# Autodesk Inventor assembly: 左後脚ユニット5_MIR
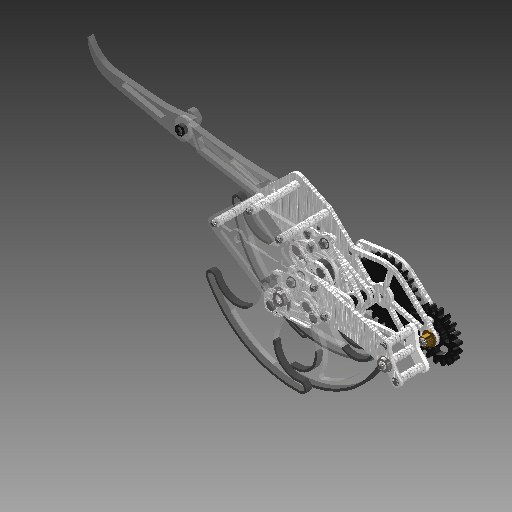
[picture p0: Inventor's stored thumbnail of the model, 512x512]
Saved by Autodesk Inventor 2020 (Build 240168000, 168)
## iProperties
Created: 2019-09-03
Part Number: 左後脚ユニット5_MIR
Document SubType Name: Assembly
Designer: 雪村
Mass: 251.015 g
Surface Area: 1556.42 cm^2
Volume: 120.818 cm^3
Density: 2.07763 g/cm^3
Author: 雪村
## Documents named in this file (29)
- C:\Users\white\Documents\SRDC\SRDC\Inventor_2017\2018年機体\2020年4年機体\右後脚ユニット5.iam
- C:\Users\white\Documents\SRDC\SRDC\Inventor_2017\2018年機体\2020年4年機体\脚内フレーム5_MIR2_MIR.ipt
- C:\Users\white\Documents\SRDC\SRDC\Inventor_2017\2018年機体\2020年4年機体\脚外フレーム5_MIR_MIR.ipt
- C:\Users\white\Documents\SRDC\SRDC\Inventor_2017\2018年機体\2020年4年機体\後脚ユニット締結パーツ5_MIR.ipt
- C:\Users\white\Documents\SRDC\SRDC\Inventor_2017\2018年機体\2020年4年機体\後脚ギアトレイン5.2_MIR.ipt
- C:\Users\white\Documents\SRDC\SRDC\Inventor_2017\2018年機体\2020年4年機体\後脚軸抑え1_MIR.ipt
- C:\Users\white\Documents\SRDC\SRDC\Inventor_2017\2018年機体\2020年4年機体\脚クランク1.iam
- C:\Users\white\Documents\SRDC\SRDC\Inventor_2017\2018年機体\2020年4年機体\ヘッケン＋揺動節2_MIR.iam
- C:\Users\white\Documents\SRDC\SRDC\Inventor_2017\2018年機体\2020年4年機体\歯車m2.z24.ipt
- C:\Users\white\Documents\SRDC\SRDC\Inventor_2017\2018年機体\2020年4年機体\脚最終段カム4.ipt
- C:\Users\white\Documents\SRDC\SRDC\Inventor_2017\2018年機体\パーツ\スペーサーm3,40.ipt
- C:\Users\white\Documents\SRDC\SRDC\Inventor_2017\2018年機体\パーツ\スペーサーm3,7.ipt
- C:\Users\white\Documents\SRDC\SRDC\Inventor_2017\2018年機体\2020年4年機体\歯車m2.z19.ipt
- C:\Users\white\Documents\SRDC\SRDC\Inventor_2017\2018年機体\パーツ\ベアリングフランジ付き0610.3t.ipt
- C:\Users\white\Documents\SRDC\SRDC\Inventor_2017\2018年機体\2020年4年機体\歯車m2.z25.ipt
- C:\Users\white\Documents\SRDC\SRDC\Inventor_2017\2018年機体\パーツ\オイレスフランジ付き06080512,1t ドライメット.ipt
- C:\Users\white\Documents\SRDC\SRDC\Inventor_2017\2018年機体\パーツ\スペーサーm3,6.ipt
- C:\Users\white\Documents\SRDC\SRDC\Inventor_2017\2018年機体\パーツ\ネジ鍋m3,12.ipt
- C:\Users\white\Documents\SRDC\SRDC\Inventor_2017\2018年機体\パーツ\オイレスフランジ付き12142003.ipt
- C:\Users\white\Documents\SRDC\SRDC\Inventor_2017\2018年機体\パーツ\スペーサーm3,4.ipt
- C:\Users\white\Documents\SRDC\SRDC\Inventor_2017\2018年機体\2020年4年機体\脚最終段カム3.ipt
- C:\Users\white\Documents\SRDC\SRDC\Inventor_2017\2018年機体\パーツ\ネジ皿m3,08.ipt
- C:\Users\white\Documents\SRDC\SRDC\Inventor_2017\2018年機体\パーツ\ネジ鍋m3,08.ipt
- C:\Users\white\Documents\SRDC\SRDC\Inventor_2017\2018年機体\パーツ\ネジ鍋m3,06.ipt
- C:\Users\white\Documents\SRDC\SRDC\Inventor_2017\2018年機体\パーツ\ネジ鍋m3,16.ipt
- C:\Users\white\Documents\SRDC\SRDC\Inventor_2017\2018年機体\2020年4年機体\後ウイング1_MIR.iam
- C:\Users\white\Documents\SRDC\SRDC\Inventor_2017\2018年機体\パーツ\スペーサーm3,20.ipt
- C:\Users\white\Documents\SRDC\SRDC\Inventor_2017\2018年機体\2020年4年機体\段ばね抑え2.ipt
- C:\Users\white\Documents\SRDC\SRDC\Inventor_2017\2018年機体\パーツ\スペーサーm3,5.ipt
## Components (75 placed, 28 different names)
1. 脚内フレーム5_MIR2_MIR:1 — メイト:1, メイト:2, メイト:3, メイト:4, 挿入:15, 挿入:16, 挿入:17, 挿入:18, 挿入:32, 挿入:33, 挿入:34, 挿入:36, 挿入:37, 挿入:38, 挿入:40, 挿入:41, 挿入:42, 挿入:44, 挿入:47, 挿入:48, 挿入:64, 挿入:70, 挿入:71, 挿入:72, 挿入:77
2. 脚外フレーム5_MIR_MIR:1 — 挿入:19, 挿入:20, 挿入:65, 挿入:66, 挿入:67, 挿入:68, 挿入:69, 挿入:90
3. 後脚ユニット締結パーツ5_MIR:1 — メイト:5, 挿入:73, 挿入:81, 挿入:82, 挿入:87, 挿入:88
4. 後脚ギアトレイン5.2_MIR:1 — 挿入:45, 挿入:46, 挿入:53, 挿入:54, 挿入:55, 挿入:62, 挿入:75
5. 後脚軸抑え1_MIR:1 — 挿入:49, 挿入:50, 挿入:56, 挿入:57, 挿入:63
6. 脚クランク1:1 [sub-assembly] — 挿入:29, メイト:6, 挿入:31, 挿入:89
7. ヘッケン＋揺動節2_MIR:1 [sub-assembly] — メイト:4
8. ヘッケン＋揺動節2_MIR:2 [sub-assembly] — メイト:3
9. ヘッケン＋揺動節2_MIR:3 [sub-assembly] — メイト:1
10. ヘッケン＋揺動節2_MIR:4 [sub-assembly] — メイト:2
11. 歯車m2.z24:1 — 挿入:30
12. 脚最終段カム4:1 — 挿入:58, 挿入:59, 挿入:60, 挿入:61
13. オイレスフランジ付き12142003:2 — メイト:7
14. スペーサーm3,40:1 — 挿入:18, 挿入:20, メイト:5
15. スペーサーm3,40:2 — 挿入:17
16. スペーサーm3,40:3 — 挿入:16
17. スペーサーm3,40:4 — 挿入:15, 挿入:19
18. スペーサーm3,7:2 — 挿入:34
19. スペーサーm3,7:3 — 挿入:38
20. スペーサーm3,7:4 — 挿入:44, 挿入:45
21. スペーサーm3,7:5 — 挿入:33, 挿入:46
22. 歯車m2.z19:1
23. ベアリングフランジ付き0610.3t:1
24. ベアリングフランジ付き0610.3t:2 — 挿入:41
25. 歯車m2.z25:1
26. ベアリングフランジ付き0610.3t:3 — 挿入:40
27. ベアリングフランジ付き0610.3t:4
28. オイレスフランジ付き06080512,1t ドライメット:1 — 挿入:75
29. オイレスフランジ付き06080512,1t ドライメット:2
30. スペーサーm3,6:1
31. スペーサーm3,6:2 — 挿入:42
32. ネジ鍋m3,12:1
33. ネジ鍋m3,12:2
34. スペーサーm3,6:3 — 挿入:37
35. スペーサーm3,6:4 — 挿入:36, 挿入:50
36. オイレスフランジ付き12142003:1 — 挿入:31, 挿入:32
37. 脚最終段カム3:1 — 挿入:29, メイト:6, 挿入:30, メイト:7
38. スペーサーm3,7:6 — 挿入:47
39. スペーサーm3,6:5 — 挿入:48, 挿入:49
40. ネジ鍋m3,12:3 — 挿入:53
41. ネジ鍋m3,12:4 — 挿入:55
42. ネジ鍋m3,12:5 — 挿入:62
43. ネジ鍋m3,12:6 — 挿入:54
44. ネジ鍋m3,12:7 — 挿入:63
45. ネジ鍋m3,12:8 — 挿入:56
46. ネジ鍋m3,12:9 — 挿入:57
47. ネジ皿m3,08:1 — 挿入:64
48. ネジ鍋m3,08:1 — 挿入:67
49. ネジ鍋m3,08:2 — 挿入:68
50. ネジ鍋m3,08:3 — 挿入:66
51. ネジ鍋m3,08:4 — 挿入:71
52. ネジ鍋m3,08:5 — 挿入:72
53. ネジ鍋m3,08:6 — 挿入:70, 挿入:76
54. ネジ鍋m3,08:7 — 挿入:69
55. ネジ鍋m3,06:1 — 挿入:65
56. ネジ鍋m3,16:1 — 挿入:61
57. ネジ鍋m3,16:2 — 挿入:59
58. ネジ鍋m3,16:3 — 挿入:60
59. ネジ鍋m3,16:4 — 挿入:58
60. スペーサーm3,4:1 — 挿入:73, 挿入:74, 挿入:86
61. ベアリングフランジ付き0610.3t:5 — 挿入:74
62. 後ウイング1_MIR:1 [sub-assembly] — 挿入:76, 正接:1
63. スペーサーm3,6:6 — 挿入:77, 正接:1
64. スペーサーm3,20:1 — 挿入:78, 挿入:82
65. スペーサーm3,20:2 — 挿入:79
66. スペーサーm3,20:3 — 挿入:80, 挿入:81
67. 段ばね抑え2:1 — 挿入:78, 挿入:79, 挿入:80, 挿入:83, 挿入:84, 挿入:85
68. ネジ鍋m3,08:8 — 挿入:84
69. ネジ鍋m3,08:9 — 挿入:83
70. ネジ鍋m3,08:10 — 挿入:85
71. ネジ鍋m3,12:10 — 挿入:86
72. ネジ皿m3,08:2 — 挿入:87
73. ネジ皿m3,08:3 — 挿入:88
74. ベアリングフランジ付き0610.3t:6 — 挿入:90
75. スペーサーm3,5:1 — 挿入:89
## Relationships (86: Insert 78, Mate 7, Tangent 1)
- [Insert] (0.5 mm): 脚クランク1:1 ↔ ヘッケン＋揺動節2_MIR:1
- [Insert] (0.5 mm): 脚クランク1:1 ↔ ヘッケン＋揺動節2_MIR:2
- [Insert] (0.5 mm): 脚クランク1:1 ↔ ヘッケン＋揺動節2_MIR:3
- [Insert] (0.5 mm): 脚クランク1:1 ↔ ヘッケン＋揺動節2_MIR:4
- [Insert]: 歯車m2.z24:1 ↔ 脚最終段カム4:1
- [Insert]: 歯車m2.z24:1 ↔ 脚最終段カム4:1
- [Insert]: 脚最終段カム4:1 ↔ オイレスフランジ付き12142003:2
- メイト:1 [Mate]: 脚内フレーム5_MIR2_MIR:1 ↔ ヘッケン＋揺動節2_MIR:3
- メイト:2 [Mate]: 脚内フレーム5_MIR2_MIR:1 ↔ ヘッケン＋揺動節2_MIR:4
- メイト:3 [Mate]: 脚内フレーム5_MIR2_MIR:1 ↔ ヘッケン＋揺動節2_MIR:2
- メイト:4 [Mate]: 脚内フレーム5_MIR2_MIR:1 ↔ ヘッケン＋揺動節2_MIR:1
- 挿入:15 [Insert]: 脚内フレーム5_MIR2_MIR:1 ↔ スペーサーm3,40:4
- 挿入:16 [Insert]: 脚内フレーム5_MIR2_MIR:1 ↔ スペーサーm3,40:3
- 挿入:17 [Insert]: 脚内フレーム5_MIR2_MIR:1 ↔ スペーサーm3,40:2
- 挿入:18 [Insert]: 脚内フレーム5_MIR2_MIR:1 ↔ スペーサーm3,40:1
- 挿入:19 [Insert]: 脚外フレーム5_MIR_MIR:1 ↔ スペーサーm3,40:4
- 挿入:20 [Insert]: 脚外フレーム5_MIR_MIR:1 ↔ スペーサーm3,40:1
- メイト:5 [Mate]: 後脚ユニット締結パーツ5_MIR:1 ↔ スペーサーm3,40:1
- [Insert]: 歯車m2.z19:1 ↔ ベアリングフランジ付き0610.3t:1
- [Insert]: 歯車m2.z19:1 ↔ ベアリングフランジ付き0610.3t:2
- [Insert]: 歯車m2.z25:1 ↔ ベアリングフランジ付き0610.3t:3
- [Insert]: 歯車m2.z25:1 ↔ ベアリングフランジ付き0610.3t:4
- [Insert]: オイレスフランジ付き06080512,1t ドライメット:1 ↔ ネジ鍋m3,12:1
- [Insert]: スペーサーm3,6:2 ↔ ネジ鍋m3,12:2
- [Insert]: オイレスフランジ付き06080512,1t ドライメット:2 ↔ スペーサーm3,6:2
- [Insert]: オイレスフランジ付き06080512,1t ドライメット:1 ↔ スペーサーm3,6:1
- 挿入:29 [Insert]: 脚クランク1:1 ↔ 脚最終段カム3:1
- メイト:6 [Mate]: 脚クランク1:1 ↔ 脚最終段カム3:1
- 挿入:30 [Insert]: 歯車m2.z24:1 ↔ 脚最終段カム3:1
- メイト:7 [Mate]: オイレスフランジ付き12142003:2 ↔ 脚最終段カム3:1
- 挿入:31 [Insert]: 脚クランク1:1 ↔ オイレスフランジ付き12142003:1
- 挿入:32 [Insert]: 脚内フレーム5_MIR2_MIR:1 ↔ オイレスフランジ付き12142003:1
- 挿入:33 [Insert]: 脚内フレーム5_MIR2_MIR:1 ↔ スペーサーm3,7:5
- 挿入:34 [Insert]: 脚内フレーム5_MIR2_MIR:1 ↔ スペーサーm3,7:2
- 挿入:36 [Insert]: 脚内フレーム5_MIR2_MIR:1 ↔ スペーサーm3,6:4
- 挿入:37 [Insert]: 脚内フレーム5_MIR2_MIR:1 ↔ スペーサーm3,6:3
- 挿入:38 [Insert]: 脚内フレーム5_MIR2_MIR:1 ↔ スペーサーm3,7:3
- 挿入:40 [Insert]: 脚内フレーム5_MIR2_MIR:1 ↔ ベアリングフランジ付き0610.3t:3
- 挿入:41 [Insert]: 脚内フレーム5_MIR2_MIR:1 ↔ ベアリングフランジ付き0610.3t:2
- 挿入:42 [Insert]: 脚内フレーム5_MIR2_MIR:1 ↔ スペーサーm3,6:2
- 挿入:44 [Insert]: 脚内フレーム5_MIR2_MIR:1 ↔ スペーサーm3,7:4
- 挿入:45 [Insert]: 後脚ギアトレイン5.2_MIR:1 ↔ スペーサーm3,7:4
- 挿入:46 [Insert]: 後脚ギアトレイン5.2_MIR:1 ↔ スペーサーm3,7:5
- 挿入:47 [Insert]: 脚内フレーム5_MIR2_MIR:1 ↔ スペーサーm3,7:6
- 挿入:48 [Insert]: 脚内フレーム5_MIR2_MIR:1 ↔ スペーサーm3,6:5
- 挿入:49 [Insert]: 後脚軸抑え1_MIR:1 ↔ スペーサーm3,6:5
- 挿入:50 [Insert]: 後脚軸抑え1_MIR:1 ↔ スペーサーm3,6:4
- 挿入:53 [Insert]: 後脚ギアトレイン5.2_MIR:1 ↔ ネジ鍋m3,12:3
- 挿入:54 [Insert]: 後脚ギアトレイン5.2_MIR:1 ↔ ネジ鍋m3,12:6
- 挿入:55 [Insert]: 後脚ギアトレイン5.2_MIR:1 ↔ ネジ鍋m3,12:4
- 挿入:56 [Insert]: 後脚軸抑え1_MIR:1 ↔ ネジ鍋m3,12:8
- 挿入:57 [Insert]: 後脚軸抑え1_MIR:1 ↔ ネジ鍋m3,12:9
- 挿入:58 [Insert]: 脚最終段カム4:1 ↔ ネジ鍋m3,16:4
- 挿入:59 [Insert]: 脚最終段カム4:1 ↔ ネジ鍋m3,16:2
- 挿入:60 [Insert]: 脚最終段カム4:1 ↔ ネジ鍋m3,16:3
- 挿入:61 [Insert]: 脚最終段カム4:1 ↔ ネジ鍋m3,16:1
- 挿入:62 [Insert]: 後脚ギアトレイン5.2_MIR:1 ↔ ネジ鍋m3,12:5
- 挿入:63 [Insert]: 後脚軸抑え1_MIR:1 ↔ ネジ鍋m3,12:7
- 挿入:64 [Insert]: 脚内フレーム5_MIR2_MIR:1 ↔ ネジ皿m3,08:1
- 挿入:65 [Insert]: 脚外フレーム5_MIR_MIR:1 ↔ ネジ鍋m3,06:1
- 挿入:66 [Insert]: 脚外フレーム5_MIR_MIR:1 ↔ ネジ鍋m3,08:3
- 挿入:67 [Insert]: 脚外フレーム5_MIR_MIR:1 ↔ ネジ鍋m3,08:1
- 挿入:68 [Insert]: 脚外フレーム5_MIR_MIR:1 ↔ ネジ鍋m3,08:2
- 挿入:69 [Insert]: 脚外フレーム5_MIR_MIR:1 ↔ ネジ鍋m3,08:7
- 挿入:70 [Insert]: 脚内フレーム5_MIR2_MIR:1 ↔ ネジ鍋m3,08:6
- 挿入:71 [Insert]: 脚内フレーム5_MIR2_MIR:1 ↔ ネジ鍋m3,08:4
- 挿入:72 [Insert]: 脚内フレーム5_MIR2_MIR:1 ↔ ネジ鍋m3,08:5
- 挿入:73 [Insert]: 後脚ユニット締結パーツ5_MIR:1 ↔ スペーサーm3,4:1
- 挿入:74 [Insert]: スペーサーm3,4:1 ↔ ベアリングフランジ付き0610.3t:5
- 挿入:75 [Insert]: 後脚ギアトレイン5.2_MIR:1 ↔ オイレスフランジ付き06080512,1t ドライメット:1
- 挿入:76 [Insert]: ネジ鍋m3,08:6 ↔ 後ウイング1_MIR:1
- 挿入:77 [Insert]: 脚内フレーム5_MIR2_MIR:1 ↔ スペーサーm3,6:6
- 挿入:78 [Insert]: スペーサーm3,20:1 ↔ 段ばね抑え2:1
- 挿入:79 [Insert]: スペーサーm3,20:2 ↔ 段ばね抑え2:1
- 挿入:80 [Insert]: スペーサーm3,20:3 ↔ 段ばね抑え2:1
- 挿入:81 [Insert]: 後脚ユニット締結パーツ5_MIR:1 ↔ スペーサーm3,20:3
- 挿入:82 [Insert]: 後脚ユニット締結パーツ5_MIR:1 ↔ スペーサーm3,20:1
- 挿入:83 [Insert]: 段ばね抑え2:1 ↔ ネジ鍋m3,08:9
- 挿入:84 [Insert]: 段ばね抑え2:1 ↔ ネジ鍋m3,08:8
- 挿入:85 [Insert]: 段ばね抑え2:1 ↔ ネジ鍋m3,08:10
- 挿入:86 [Insert]: スペーサーm3,4:1 ↔ ネジ鍋m3,12:10
- 挿入:87 [Insert]: 後脚ユニット締結パーツ5_MIR:1 ↔ ネジ皿m3,08:2
- 挿入:88 [Insert]: 後脚ユニット締結パーツ5_MIR:1 ↔ ネジ皿m3,08:3
- 正接:1 [Tangent]: 後ウイング1_MIR:1 ↔ スペーサーm3,6:6
- 挿入:89 [Insert]: 脚クランク1:1 ↔ スペーサーm3,5:1
- 挿入:90 [Insert]: 脚外フレーム5_MIR_MIR:1 ↔ ベアリングフランジ付き0610.3t:6
## Named parameters: d6_d1 = 0 mm, d7_d0 = 0 mm, d43_d9 = 0 mm, d44_d10 = 0 mm, d42_d20 = 0 mm, d43_d21 = 0 mm, d44_d17 = 0 mm, d45_d19 = 0 mm
